# Autodesk Inventor assembly: Linear Slide Assembly
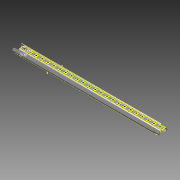
[picture p0: Inventor's stored thumbnail of the model, 180x180]
Saved by Autodesk Inventor 2014 (Build 180170000, 170)
## iProperties
Created: 2010-08-13
Part Number: Linear Slide Assembly
Document SubType Name: Assembly
Designer: Hannah
Translation Standard: STEP AP203
FileName: Linear Slide Assembly.iam
PreProcessor: SolidWorks 2007
PostProcessor: Build: 239, Release: 2011 RTM - Date: Wed 02/17/2010
Sent Units: inch
Uncertainty: 1e-05
Author: Hannah
## Documents named in this file (3)
- F:\Inventor\Robotics\Vex parts\Metal Other\Linear Slide Assembly.iam
- F:\Inventor\Robotics\Vex parts\Metal Other\Linear Slide Assembly-Parts\Linear Slide-Inner.ipt
- F:\Inventor\Robotics\Vex parts\Metal Other\Linear Slide Assembly-Parts\Linear Slide-Outer.ipt
## Components (2 placed, 2 different names)
1. Linear Slide-Outer:1 — Mate:1, Flush:1
2. Linear Slide-Inner:1 — Mate:1, Flush:1
## Relationships (2: Mate 1, Flush 1)
- Mate:1 (10.16 mm): Linear Slide-Outer:1 ↔ Linear Slide-Inner:1
- Flush:1: Linear Slide-Outer:1 ↔ Linear Slide-Inner:1
